# Autodesk Inventor assembly: LandingGear
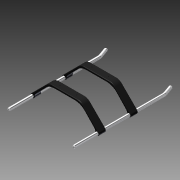
[picture p0: Inventor's stored thumbnail of the model, 180x180]
Saved by Autodesk Inventor 2011 SP1 (Build 150282100, 282)
## iProperties
Created: 2011-08-02
Part Number: LandingGear
Document SubType Name: Assembly
Designer: Nathan
Author: Nathan
## Documents named in this file (3)
- C:\Users\Nathan\Documents\Inventor\Quadcopter\LandingGear.iam
- C:\Users\Nathan\Documents\Inventor\Quadcopter\LandingBracket.ipt
- C:\Users\Nathan\Documents\Inventor\Quadcopter\LandingSkid.ipt
## Components (4 placed, 2 different names)
1. LandingBracket:1 — Mate:1, Mate:3, Mate:5
2. LandingBracket:2 — Mate:2, Mate:4, Mate:5, Angle:1, Angle:2
3. LandingSkid:1 — Mate:1, Mate:2, Flush:1, Angle:2
4. LandingSkid:2 — Mate:3, Mate:4, Flush:1, Angle:1
## Relationships (8: Mate 5, Angle 2, Flush 1)
- Mate:1: LandingBracket:1 ↔ LandingSkid:1
- Mate:2: LandingBracket:2 ↔ LandingSkid:1
- Mate:3: LandingBracket:1 ↔ LandingSkid:2
- Mate:4: LandingBracket:2 ↔ LandingSkid:2
- Flush:1: LandingSkid:1 ↔ LandingSkid:2
- Mate:5 (101.6 mm): LandingBracket:1 ↔ LandingBracket:2
- Angle:1 (0 deg): LandingBracket:2 ↔ LandingSkid:2
- Angle:2 (0 deg): LandingBracket:2 ↔ LandingSkid:1
